# Autodesk Inventor assembly: Dispensador
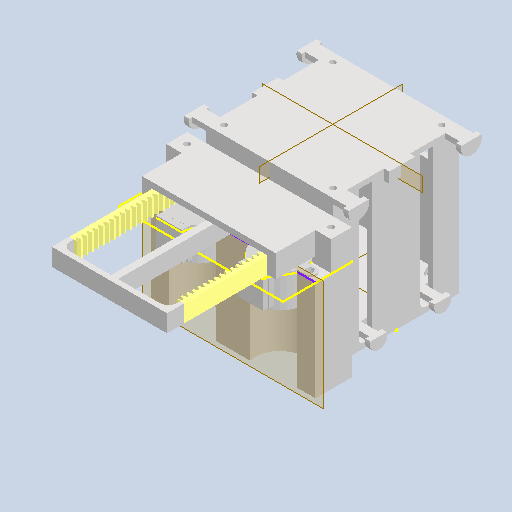
[picture p0: Inventor's stored thumbnail of the model, 512x512]
Saved by Autodesk Inventor 2024 (Build 280153000, 153)
## iProperties
Created: 2025-03-02
Part Number: Dispensador
Document SubType Name: Assembly
Designer: sergi
Author: sergi
## Documents named in this file (9)
- C:\Users\sergi\OneDrive\Escritorio\Projects\16. Protection catapult\Inventor\Dispensador.iam
- C:\Users\sergi\OneDrive\Escritorio\Projects\16. Protection catapult\Inventor\Base dispensador.ipt
- C:\Users\sergi\OneDrive\Escritorio\Projects\16. Protection catapult\Inventor\Tapa dispensador.ipt
- C:\Users\sergi\OneDrive\Escritorio\Projects\16. Protection catapult\Inventor\Parte deslizante.ipt
- C:\Users\sergi\OneDrive\Escritorio\Projects\16. Protection catapult\Inventor\igus_20250223_174552\StepMotor28BYJ.ipt
- C:\Users\sergi\OneDrive\Escritorio\Projects\16. Protection catapult\Inventor\igus_20250223_174552\10301_para_engranajes_1\10301_para_engranajes_1.ipt
- C:\Users\sergi\OneDrive\Escritorio\Projects\16. Protection catapult\Inventor\Cremallera.iam
- C:\Users\sergi\OneDrive\Escritorio\Projects\16. Protection catapult\Inventor\Base Motores.ipt
- C:\Users\sergi\OneDrive\Escritorio\Projects\16. Protection catapult\Inventor\Tapadera cremallera.ipt
## Components (10 placed, 8 different names)
1. Base dispensador:1 — Nivelación:1, Coincidencia:1, Coincidencia:2, Coincidencia:3, Nivelación:2, Nivelación:3, Ángulo:1, Ángulo:2, Coincidencia:10, Coincidencia:11, Coincidencia:12, Nivelación:7
2. Tapa dispensador:1 — Nivelación:1
3. Parte deslizante:1 — Coincidencia:1, Coincidencia:2, Coincidencia:3
4. StepMotor28BYJ:1 — Nivelación:2, Ángulo:1, Nivelación:4, Coincidencia:8
5. StepMotor28BYJ:2 — Nivelación:3, Ángulo:2, Nivelación:4, Coincidencia:4, Coincidencia:10
6. 10301_para_engranajes_1:1 — Coincidencia:4, Coincidencia:13, Nivelación:5, Rotación/Traslación:1
7. Cremallera:1 [sub-assembly] — Coincidencia:11, Coincidencia:12, Coincidencia:13, Nivelación:5, Nivelación:6, Coincidencia:14, Rotación/Traslación:1, Rotación/Traslación:2
8. 10301_para_engranajes_1:2 — Coincidencia:8, Nivelación:6, Coincidencia:14, Rotación/Traslación:2
9. Base Motores:1 — Nivelación:7, Nivelación:8
10. Tapadera cremallera:1 — Nivelación:8
## Relationships (22: Mate 10, Flush 8, Angle 2, RelateRotateTranslate 2)
- Nivelación:1 [Flush]: Base dispensador:1 ↔ Tapa dispensador:1
- Coincidencia:1 [Mate] (4 mm): Base dispensador:1 ↔ Parte deslizante:1
- Coincidencia:2 [Mate] (1.5 mm): Base dispensador:1 ↔ Parte deslizante:1
- Coincidencia:3 [Mate] (1.5 mm): Base dispensador:1 ↔ Parte deslizante:1
- Nivelación:2 [Flush] (2 mm): Base dispensador:1 ↔ StepMotor28BYJ:1
- Nivelación:3 [Flush] (2 mm): Base dispensador:1 ↔ StepMotor28BYJ:2
- Ángulo:1 [Angle] (0 deg): Base dispensador:1 ↔ StepMotor28BYJ:1
- Ángulo:2 [Angle] (0 deg): Base dispensador:1 ↔ StepMotor28BYJ:2
- Nivelación:4 [Flush]: StepMotor28BYJ:1 ↔ StepMotor28BYJ:2
- Coincidencia:4 [Mate]: StepMotor28BYJ:2 ↔ 10301_para_engranajes_1:1
- Coincidencia:8 [Mate]: StepMotor28BYJ:1 ↔ 10301_para_engranajes_1:2
- Coincidencia:10 [Mate] (17.5 mm): Base dispensador:1 ↔ StepMotor28BYJ:2
- Coincidencia:11 [Mate] (0.3 mm): Base dispensador:1 ↔ Cremallera:1
- Coincidencia:12 [Mate]: Base dispensador:1 ↔ Cremallera:1
- Coincidencia:13 [Mate] (7.5 mm): 10301_para_engranajes_1:1 ↔ Cremallera:1
- Nivelación:5 [Flush]: 10301_para_engranajes_1:1 ↔ Cremallera:1
- Nivelación:6 [Flush]: Cremallera:1 ↔ 10301_para_engranajes_1:2
- Coincidencia:14 [Mate] (7.5 mm): Cremallera:1 ↔ 10301_para_engranajes_1:2
- Rotación/Traslación:1 [RelateRotateTranslate] (15.708 mm): 10301_para_engranajes_1:1 ↔ Cremallera:1
- Rotación/Traslación:2 [RelateRotateTranslate] (15.708 mm): Cremallera:1 ↔ 10301_para_engranajes_1:2
- Nivelación:7 [Flush]: Base dispensador:1 ↔ Base Motores:1
- Nivelación:8 [Flush]: Base Motores:1 ↔ Tapadera cremallera:1
